# Autodesk Inventor assembly: roughDraft-12inchBase
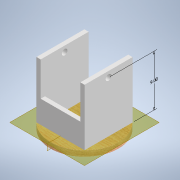
[picture p0: Inventor's stored thumbnail of the model, 180x180]
Saved by Autodesk Inventor 2022.2 (Build 262287000, 287)
## iProperties
Created: 2020-07-01
Part Number: roughDraft-12inchBase
Document SubType Name: Assembly
Designer: robst
Author: robst
## Documents named in this file (5)
- C:\git\CAD-Development\robSteele\ShapeWays\TelescopeProjects\TelescopeMount\roughDraft-12inchBase.iam
- C:\git\CAD-Development\robSteele\ShapeWays\TelescopeProjects\TelescopeMount\base-12-inch-diameter.ipt
- C:\git\CAD-Development\robSteele\ShapeWays\TelescopeProjects\TelescopeMount\sideSupportFor12inchBase.ipt
- C:\git\CAD-Development\robSteele\ShapeWays\TelescopeProjects\TelescopeMount\sideSupportFor12inchBase_MIR.ipt
- C:\git\CAD-Development\robSteele\ShapeWays\TelescopeProjects\TelescopeMount\frontSupportFor12inchBase.ipt
## Components (4 placed, 4 different names)
1. base-12-inch-diameter:1 — Flush:1, Flush:2, Flush:3, Flush:4
2. sideSupportFor12inchBase:1 — Flush:1, Flush:2
3. sideSupportFor12inchBase_MIR:1
4. frontSupportFor12inchBase:1 — Flush:3, Flush:4
## Relationships (4: Flush 4)
- Flush:1: base-12-inch-diameter:1 ↔ sideSupportFor12inchBase:1
- Flush:2: base-12-inch-diameter:1 ↔ sideSupportFor12inchBase:1
- Flush:3: base-12-inch-diameter:1 ↔ frontSupportFor12inchBase:1
- Flush:4: base-12-inch-diameter:1 ↔ frontSupportFor12inchBase:1
